# Autodesk Inventor assembly: Master Assembly
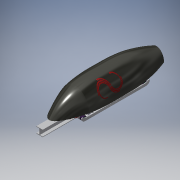
[picture p0: Inventor's stored thumbnail of the model, 180x180]
Saved by Autodesk Inventor 2018 (Build 220112000, 112)
## iProperties
Created: 2017-10-11
Part Number: Master Assembly
Document SubType Name: Assembly
Designer: cxa2
Mass: 1.13635e+06 g
Surface Area: 545760 cm^2
Volume: 1.09483e+06 cm^3
Density: 1.03793 g/cm^3
Author: cxa2
## Documents named in this file (23)
- E:\Hyperloop Full CAD\Master Assembly.iam
- C:\Users\jt665\Documents\Vault\Hyperloop2018\Master Assembly\Track Parts\Tube.ipt
- C:\Users\jt665\Documents\Vault\Hyperloop2018\Master Assembly\Track Parts\I-Beam.ipt
- C:\Users\jt665\Documents\Vault\Hyperloop2018\Master Assembly\Track Parts\Subtrack.ipt
- C:\Users\jt665\Documents\Vault\Hyperloop2018\Suspension\Rail Follower\FOLLOWRAIL.iam
- C:\Users\jt665\Documents\Vault\Hyperloop2018\Suspension\Ski & Shocks\Ski Assembly.iam
- C:\Users\jt665\Documents\Vault\Hyperloop2018\Suspension\Chassis\Chassis.iam
- C:\Users\jt665\Documents\Vault\Hyperloop2018\Suspension\Rail Follower\FOLLOWRAIL_2.iam
- C:\Users\jt665\Documents\Vault\Hyperloop2018\Fuselage\Shell\Pod Shell.ipt
- C:\Users\jt665\Documents\Vault\Hyperloop2018\Suspension\Brakes\CubeBrake.iam
- C:\Users\jt665\Documents\Vault\Hyperloop2018\Fuselage\Propulsion System\Valves\EH40 Solenoid.ipt
- C:\Users\jt665\Documents\Vault\Hyperloop2018\Fuselage\Propulsion System\Valves\H2B-M-12N-S316.iam
- C:\Users\jt665\Documents\Vault\Hyperloop2018\Fuselage\Propulsion System\Valves\H1B-M-8N-S316.iam
- C:\Users\jt665\Documents\Vault\Hyperloop2018\Fuselage\Propulsion System\Tanks\Luxfer_T188C_Estimate.ipt
- C:\Users\jt665\Documents\Vault\Hyperloop2018\Fuselage\Propulsion System\Tank Holder\Tank Holder Assembly.iam
- C:\Users\jt665\Documents\Vault\Hyperloop2018\Fuselage\Propulsion System\Valves\Restriction Orifice Estimate.ipt
- C:\Users\jt665\Documents\Vault\Hyperloop2018\Fuselage\Propulsion System\Valves\Parts\Ball Valve Holder.ipt
- C:\Users\jt665\Documents\Vault\Hyperloop2018\Fuselage\Propulsion System\Valves\Parts\Straight Hose.ipt
- C:\Users\jt665\Documents\Vault\Hyperloop2018\Fuselage\Propulsion System\Valves\Parts\Orifice Holder.ipt
- C:\Users\jt665\Documents\Vault\Hyperloop2018\Fuselage\Propulsion System\Valves\Parts\Solenoid Holder.ipt
- C:\Users\jt665\Documents\Vault\Hyperloop2018\Fuselage\Propulsion System\Load Path.ipt
- C:\Users\jt665\Documents\Vault\Hyperloop2018\Master Assembly\Master Assembly\AIP\Tube and Pipe\Master Assembly.Tube and Pipe Runs01.iam
- C:\Users\jt665\Documents\Vault\Hyperloop2018\Fuselage\Nozzle 1-26.ipt
## Components (34 placed, 22 different names)
1. Tube:1 — Mate:1, Flush:1, Mate:2, Flush:13
2. I-Beam:1 — Mate:3, Flush:2, Mate:4, Angle:4, Mate:11, Mate:13, Angle:7, Angle:9, Angle:10, Mate:14, Mate:17, Angle:11, Angle:12, Angle:13, Mate:19, Mate:24
3. Subtrack:1 — Mate:5, Flush:3, Mate:6, Angle:5, Mate:7, Mate:8, Angle:8, Mate:16
4. FOLLOWRAIL:1 [sub-assembly] — Mate:13, Angle:7, Angle:8, Flush:5, Flush:6, Mate:40, Mate:46
5. FOLLOWRAIL:3 [sub-assembly] — Angle:9, Angle:10, Mate:14, Flush:4, Mate:22, Mate:47
6. Ski Assembly:1 [sub-assembly] — Mate:8, Mate:37, Mate:38, Mate:39
7. Ski Assembly:2 [sub-assembly] — Angle:4, Angle:5, Mate:7, Mate:11, Mate:37, Mate:38, Mate:39, Mate:40
8. Chassis:1 [sub-assembly] — Mate:16, Mate:17, Flush:6, Flush:8, Flush:9, Flush:13, Mate:45, Mate:46, Mate:47, Mate:48, Mate:49, Mate:50, Mate:51, Mate:52, Mate:53, Flush:14, Mate:54, Flush:15, Mate:55, Mate:56, Flush:16, Flush:20, Mate:62, Mate:63, Mate:64, Mate:65, Mate:68, Mate:69, Flush:22, Mate:75, Flush:23, Mate:76
9. FOLLOWRAIL_2:1 [sub-assembly] — Angle:12, Flush:5, Mate:22, Mate:24, Mate:45
10. FOLLOWRAIL_2:2 [sub-assembly] — Angle:11, Angle:13, Mate:19, Flush:4, Mate:48
11. Pod Shell:1 — Flush:7, Flush:8, Flush:9, Flush:16
12. Nozzle 1-26:1 — Insert:14
13. Nozzle 1-26:2 — Insert:15
14. CubeBrake:1 [sub-assembly] — Mate:49, Mate:50
15. CubeBrake:2 [sub-assembly] — Mate:51, Mate:52
16. EH40 Solenoid:1 — Insert:12, Mate:70
17. EH40 Solenoid:2 — Insert:11, Mate:71
18. H2B-M-12N-S316:1 [sub-assembly] — Insert:3
19. H2B-M-12N-S316:2 [sub-assembly] — Insert:4
20. H1B-M-8N-S316:1 [sub-assembly] — Mate:57, Mate:58, Flush:17, Insert:10
21. H1B-M-8N-S316:2 [sub-assembly] — Mate:59, Flush:18, Mate:60, Insert:9
22. Luxfer_T188C_Estimate:1 — Insert:1, Insert:4
23. Luxfer_T188C_Estimate:2 — Insert:2, Insert:3
24. Tank Holder Assembly:1 [sub-assembly] — Mate:54, Flush:15, Mate:55
25. Tank Holder Assembly:2 [sub-assembly] — Mate:53, Flush:14, Mate:56, Insert:1, Insert:2
26. Restriction Orifice Estimate:1 — Insert:8
27. Restriction Orifice Estimate:2 — Insert:7
28. Ball Valve Holder:1 — Mate:57, Mate:58, Flush:17, Mate:59, Flush:18, Mate:60, Flush:20, Mate:62, Mate:63
29. Straight Hose:1 — Insert:8, Insert:10
30. Straight Hose:2 — Insert:7, Insert:9, Flush:21
31. Orifice Holder:1 — Mate:64, Mate:65, Flush:21
32. Solenoid Holder:1 — Mate:68, Mate:69, Insert:11, Insert:12, Mate:70, Mate:71, Flush:22
33. Load Path:1 — Mate:75, Flush:23, Mate:76, Insert:14, Insert:15
34. Tube & Pipe Runs 01 [sub-assembly]
## Relationships (88: Mate 47, Flush 19, Insert 13, Angle 9)
- Mate:1: Tube:1
- Flush:1: Tube:1
- Mate:2: Tube:1
- Mate:3: I-Beam:1
- Flush:2: I-Beam:1
- Mate:4: I-Beam:1
- Mate:5: Subtrack:1
- Flush:3: Subtrack:1
- Mate:6: Subtrack:1
- Angle:4 (0 deg): I-Beam:1 ↔ Ski Assembly:2
- Angle:5 (0 deg): Subtrack:1 ↔ Ski Assembly:2
- Mate:7 (40.005 mm): Subtrack:1 ↔ Ski Assembly:2
- Mate:8 (40.005 mm): Subtrack:1 ↔ Ski Assembly:1
- Mate:11 (76.2 mm): I-Beam:1 ↔ Ski Assembly:2
- Mate:13 (55.118 mm): I-Beam:1 ↔ FOLLOWRAIL:1
- Angle:7 (180 deg): I-Beam:1 ↔ FOLLOWRAIL:1
- Angle:8 (180 deg): Subtrack:1 ↔ FOLLOWRAIL:1
- Angle:9 (180 deg): I-Beam:1 ↔ FOLLOWRAIL:3
- Angle:10 (0 deg): I-Beam:1 ↔ FOLLOWRAIL:3
- Mate:14 (55.118 mm): I-Beam:1 ↔ FOLLOWRAIL:3
- Mate:16 (127.254 mm): Subtrack:1 ↔ Chassis:1
- Mate:17 (95.25 mm): I-Beam:1 ↔ Chassis:1
- Angle:11 (0 deg): I-Beam:1 ↔ FOLLOWRAIL_2:2
- Angle:12 (0 deg): I-Beam:1 ↔ FOLLOWRAIL_2:1
- Angle:13 (180 deg): I-Beam:1 ↔ FOLLOWRAIL_2:2
- Mate:19 (55.118 mm): I-Beam:1 ↔ FOLLOWRAIL_2:2
- Flush:4: FOLLOWRAIL:3 ↔ FOLLOWRAIL_2:2
- Flush:5: FOLLOWRAIL:1 ↔ FOLLOWRAIL_2:1
- Mate:22 (762 mm): FOLLOWRAIL:3 ↔ FOLLOWRAIL_2:1
- Mate:24 (55.118 mm): I-Beam:1 ↔ FOLLOWRAIL_2:1
- Flush:6 (88.9 mm): FOLLOWRAIL:1 ↔ Chassis:1
- Flush:7: Pod Shell:1
- Flush:8: Chassis:1 ↔ Pod Shell:1
- Flush:9 (-266.7 mm): Chassis:1 ↔ Pod Shell:1
- Flush:13 (508 mm): Tube:1 ↔ Chassis:1
- Mate:37: Ski Assembly:1 ↔ Ski Assembly:2
- Mate:38: Ski Assembly:1 ↔ Ski Assembly:2
- Mate:39 (279.4 mm): Ski Assembly:1 ↔ Ski Assembly:2
- Mate:40: FOLLOWRAIL:1 ↔ Ski Assembly:2
- Mate:45: Chassis:1 ↔ FOLLOWRAIL_2:1
- Mate:46: FOLLOWRAIL:1 ↔ Chassis:1
- Mate:47: FOLLOWRAIL:3 ↔ Chassis:1
- Mate:48: Chassis:1 ↔ FOLLOWRAIL_2:2
- Mate:49: Chassis:1 ↔ CubeBrake:1
- Mate:50: Chassis:1 ↔ CubeBrake:1
- Mate:51: Chassis:1 ↔ CubeBrake:2
- Mate:52: Chassis:1 ↔ CubeBrake:2
- Mate:53: Chassis:1 ↔ Tank Holder Assembly:2
- Flush:14: Chassis:1 ↔ Tank Holder Assembly:2
- Mate:54: Chassis:1 ↔ Tank Holder Assembly:1
- Flush:15: Chassis:1 ↔ Tank Holder Assembly:1
- Mate:55 (101.6 mm): Chassis:1 ↔ Tank Holder Assembly:1
- Mate:56 (101.6 mm): Chassis:1 ↔ Tank Holder Assembly:2
- Insert:1 (330.2 mm): Luxfer_T188C_Estimate:1 ↔ Tank Holder Assembly:2
- Insert:2 (330.2 mm): Luxfer_T188C_Estimate:2 ↔ Tank Holder Assembly:2
- Insert:3: H2B-M-12N-S316:1 ↔ Luxfer_T188C_Estimate:2
- Insert:4: H2B-M-12N-S316:2 ↔ Luxfer_T188C_Estimate:1
- Flush:16 (25.4 mm): Chassis:1 ↔ Pod Shell:1
- Mate:57: H1B-M-8N-S316:1 ↔ Ball Valve Holder:1
- Mate:58: H1B-M-8N-S316:1 ↔ Ball Valve Holder:1
- Flush:17: H1B-M-8N-S316:1 ↔ Ball Valve Holder:1
- Mate:59: H1B-M-8N-S316:2 ↔ Ball Valve Holder:1
- Flush:18: H1B-M-8N-S316:2 ↔ Ball Valve Holder:1
- Mate:60: H1B-M-8N-S316:2 ↔ Ball Valve Holder:1
- Flush:20 (-254 mm): Chassis:1 ↔ Ball Valve Holder:1
- Insert:7: Restriction Orifice Estimate:2 ↔ Straight Hose:2
- Insert:8: Restriction Orifice Estimate:1 ↔ Straight Hose:1
- Insert:9: H1B-M-8N-S316:2 ↔ Straight Hose:2
- Insert:10: H1B-M-8N-S316:1 ↔ Straight Hose:1
- Mate:62: Chassis:1 ↔ Ball Valve Holder:1
- Mate:63: Chassis:1 ↔ Ball Valve Holder:1
- Mate:64: Chassis:1 ↔ Orifice Holder:1
- Mate:65: Chassis:1 ↔ Orifice Holder:1
- Flush:21: Straight Hose:2 ↔ Orifice Holder:1
- Mate:68: Chassis:1 ↔ Solenoid Holder:1
- Mate:69: Chassis:1 ↔ Solenoid Holder:1
- Insert:11: EH40 Solenoid:2 ↔ Solenoid Holder:1
- Insert:12: EH40 Solenoid:1 ↔ Solenoid Holder:1
- Mate:70: EH40 Solenoid:1 ↔ Solenoid Holder:1
- Mate:71: EH40 Solenoid:2 ↔ Solenoid Holder:1
- Flush:22 (-88.9 mm): Chassis:1 ↔ Solenoid Holder:1
- [Mate]: Nozzle 1-26:1 ↔ Load Path:1
- [Insert]: Nozzle 1-26:1 ↔ Load Path:1
- Mate:75: Chassis:1 ↔ Load Path:1
- Flush:23: Chassis:1 ↔ Load Path:1
- Mate:76: Chassis:1 ↔ Load Path:1
- Insert:14: Nozzle 1-26:1 ↔ Load Path:1
- Insert:15: Nozzle 1-26:2 ↔ Load Path:1
